# Autodesk Inventor assembly: pcb_assembled_2
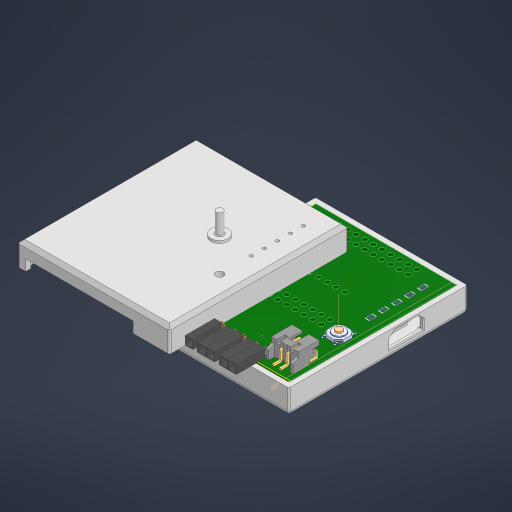
[picture p0: Inventor's stored thumbnail of the model, 512x512]
Saved by Autodesk Inventor 2023 (Build 270158000, 158)
## iProperties
Created: 2022-04-29
Part Number: pcb_assembled_2
Document SubType Name: Assembly
Designer: Haroon Nawaz
Author: Haroon Nawaz
## Documents named in this file (6)
- C:\Users\Haroon Nawaz\Documents\1_Haroon\CE347\git\CE347_Gest\hardware\3D_CAD\pcb_assembled_3.iam
- C:\Users\Haroon Nawaz\Documents\1_Haroon\CE347\git\CE347_Gest\hardware\3D_CAD\pcb_assembled.iam
- C:\Users\Haroon Nawaz\Documents\1_Haroon\CE347\git\CE347_Gest\hardware\3D_CAD\battery.ipt
- C:\Users\Haroon Nawaz\Documents\1_Haroon\CE347\git\CE347_Gest\hardware\3D_CAD\enclosure3.ipt
- C:\Users\Haroon Nawaz\Documents\1_Haroon\CE347\git\CE347_Gest\hardware\3D_CAD\enclosure3_top.ipt
- C:\Users\Haroon Nawaz\Documents\1_Haroon\CE347\git\CE347_Gest\hardware\3D_CAD\enclosure3_button.ipt
## Components (5 placed, 5 different names)
1. pcb_assembled:1 [sub-assembly] — Mate:3, Flush:1, Flush:2, Mate:4
2. battery:1 — Mate:3
3. enclosure3:1 — Flush:1, Flush:2, Mate:4
4. enclosure3_top:1 — Mate:7
5. enclosure3_button:1 — Mate:7
## Relationships (5: Mate 3, Flush 2)
- Mate:3: pcb_assembled:1 ↔ battery:1
- Flush:1 (1.55 mm): pcb_assembled:1 ↔ enclosure3:1
- Flush:2 (1.55 mm): pcb_assembled:1 ↔ enclosure3:1
- Mate:4: pcb_assembled:1 ↔ enclosure3:1
- Mate:7: enclosure3_top:1 ↔ enclosure3_button:1
